# Autodesk Inventor assembly: Assembly1
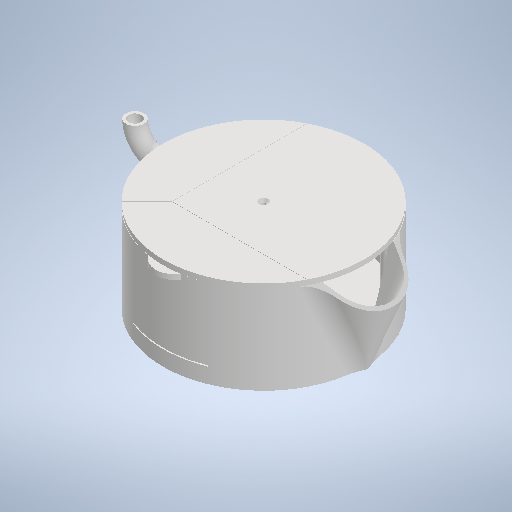
[picture p0: Inventor's stored thumbnail of the model, 512x512]
Saved by Autodesk Inventor 2025 (Build 290162000, 162)
## iProperties
Created: 2026-03-19
Part Number: Assembly1
Document SubType Name: Assembly
Designer: Luca
Author: Luca
## Documents named in this file (12)
- C:\Users\Luca\Documents\Inventor\Pflanzen\Assembly1.iam
- C:\Users\Luca\Documents\Inventor\Pflanzen\reservoir.ipt
- C:\Users\Luca\Documents\Inventor\Pflanzen\left_hull.ipt
- C:\Users\Luca\Documents\Inventor\Pflanzen\bottom_hull.ipt
- C:\Users\Luca\Documents\Inventor\Pflanzen\bottom_hull_lid.ipt
- C:\Users\Luca\Documents\Inventor\Pflanzen\left_hull_lid.ipt
- C:\Users\Luca\Documents\Inventor\Pflanzen\reservoir_lid.ipt
- C:\Users\Luca\Documents\Inventor\Pflanzen\battery_lid.ipt
- C:\Users\Luca\Documents\Inventor\Pflanzen\pipe_angle.ipt
- C:\Users\Luca\Documents\Inventor\Pflanzen\secrure_ring.ipt
- C:\Users\Luca\Documents\Inventor\Pflanzen\button.ipt
- C:\Users\Luca\Documents\Inventor\Pflanzen\button_mount.ipt
## Components (11 placed, 11 different names)
1. reservoir:1 — Mate:1, Mate:2, Mate:3, Mate:4, Mate:5, Mate:6, Mate:13, Mate:14, Mate:15
2. left_hull:1 — Mate:1, Mate:2, Mate:3, Mate:10, Mate:11, Mate:12, Mate:20, Mate:21, Mate:22, Mate:23, Mate:24, Mate:25
3. bottom_hull:1 — Mate:4, Mate:5, Mate:6, Mate:7, Mate:8, Mate:9, Mate:17, Mate:18
4. bottom_hull_lid:1 — Mate:7, Mate:8, Mate:9, Mate:27
5. left_hull_lid:1 — Mate:10, Mate:11, Mate:12
6. reservoir_lid:1 — Mate:13, Mate:14, Mate:15
7. battery_lid:1 — Mate:27, Mate:17, Mate:18
8. pipe_angle:1 — Mate:19, Mate:20, Mate:21, Flush:1
9. secrure_ring:1 — Mate:19, Flush:1
10. button:1 — Mate:24, Mate:25, Mate:26
11. button_mount:1 — Mate:22, Mate:23, Mate:26
## Relationships (27: Mate 26, Flush 1)
- Mate:1: reservoir:1 ↔ left_hull:1
- Mate:2: reservoir:1 ↔ left_hull:1
- Mate:3 (0.1 mm): reservoir:1 ↔ left_hull:1
- Mate:4: reservoir:1 ↔ bottom_hull:1
- Mate:5: reservoir:1 ↔ bottom_hull:1
- Mate:6 (0.1 mm): reservoir:1 ↔ bottom_hull:1
- Mate:7: bottom_hull:1 ↔ bottom_hull_lid:1
- Mate:8: bottom_hull:1 ↔ bottom_hull_lid:1
- Mate:9: bottom_hull:1 ↔ bottom_hull_lid:1
- Mate:10: left_hull:1 ↔ left_hull_lid:1
- Mate:11: left_hull:1 ↔ left_hull_lid:1
- Mate:12: left_hull:1 ↔ left_hull_lid:1
- Mate:13: reservoir:1 ↔ reservoir_lid:1
- Mate:14: reservoir:1 ↔ reservoir_lid:1
- Mate:15: reservoir:1 ↔ reservoir_lid:1
- Mate:27: bottom_hull_lid:1 ↔ battery_lid:1
- Mate:17 (0.25 mm): bottom_hull:1 ↔ battery_lid:1
- Mate:18 (0.25 mm): bottom_hull:1 ↔ battery_lid:1
- Mate:19: pipe_angle:1 ↔ secrure_ring:1
- Mate:20: left_hull:1 ↔ pipe_angle:1
- Mate:21: left_hull:1 ↔ pipe_angle:1
- Flush:1: pipe_angle:1 ↔ secrure_ring:1
- Mate:22: left_hull:1 ↔ button_mount:1
- Mate:23 (0.1 mm): left_hull:1 ↔ button_mount:1
- Mate:24: left_hull:1 ↔ button:1
- Mate:25 (0.1 mm): left_hull:1 ↔ button:1
- Mate:26 (5 mm): button:1 ↔ button_mount:1
